# Autodesk Inventor assembly: chassis_2
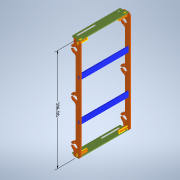
[picture p0: Inventor's stored thumbnail of the model, 180x180]
Saved by Autodesk Inventor 2022 (Build 260153000, 153)
## iProperties
Created: 2023-03-24
Part Number: chassis_2
Document SubType Name: Assembly
Designer: Johnny Jou
Author: Johnny Jou
## Documents named in this file (5)
- C:\Users\Johnny Jou\Documents\GitHub\Areo_Rider_Cabin\car\chassis_2.iam
- C:\Users\Johnny Jou\Documents\GitHub\Areo_Rider_Cabin\car\chassis_1_1.ipt
- C:\Users\Johnny Jou\Documents\GitHub\Areo_Rider_Cabin\car\chassis_1_2.ipt
- C:\Users\Johnny Jou\Documents\GitHub\Areo_Rider_Cabin\car\chassis_1_3.ipt
- C:\Users\Johnny Jou\Documents\GitHub\Areo_Rider_Cabin\car\chassis_1_4.ipt
## Components (10 placed, 4 different names)
1. chassis_1_1:1 — 貼合:1, 齊平:1, 齊平:2, 貼合:3, 貼合:4, 貼合:6, 齊平:5, 貼合:7, 貼合:8, 齊平:6, 貼合:9, 齊平:8, 齊平:12
2. chassis_1_1:2 — 貼合:2, 貼合:5, 齊平:4, 齊平:9, 齊平:15
3. chassis_1_2:1 — 貼合:1, 齊平:2, 齊平:3, 貼合:10, 齊平:7, 齊平:10
4. chassis_1_2:2 — 貼合:2, 齊平:1, 齊平:3, 貼合:3, 貼合:4, 貼合:5, 齊平:4, 貼合:11, 齊平:13, 齊平:16
5. chassis_1_3:1 — 貼合:6, 齊平:5, 貼合:7
6. chassis_1_3:2 — 貼合:8, 齊平:6, 貼合:9
7. chassis_1_4:1 — 貼合:10, 齊平:7, 齊平:8, 齊平:11
8. chassis_1_4:2 — 齊平:9, 齊平:10, 齊平:11
9. chassis_1_4:3 — 貼合:11, 齊平:12, 齊平:13, 齊平:14
10. chassis_1_4:4 — 齊平:14, 齊平:15, 齊平:16
## Relationships (27: Flush 16, Mate 11)
- 貼合:1 [Mate]: chassis_1_1:1 ↔ chassis_1_2:1
- 貼合:2 [Mate]: chassis_1_1:2 ↔ chassis_1_2:2
- 齊平:1 [Flush]: chassis_1_1:1 ↔ chassis_1_2:2
- 齊平:2 [Flush]: chassis_1_1:1 ↔ chassis_1_2:1
- 齊平:3 [Flush]: chassis_1_2:1 ↔ chassis_1_2:2
- 貼合:3 [Mate]: chassis_1_1:1 ↔ chassis_1_2:2
- 貼合:4 [Mate]: chassis_1_1:1 ↔ chassis_1_2:2
- 貼合:5 [Mate]: chassis_1_1:2 ↔ chassis_1_2:2
- 齊平:4 [Flush]: chassis_1_1:2 ↔ chassis_1_2:2
- 貼合:6 [Mate]: chassis_1_1:1 ↔ chassis_1_3:1
- 齊平:5 [Flush]: chassis_1_1:1 ↔ chassis_1_3:1
- 貼合:7 [Mate]: chassis_1_1:1 ↔ chassis_1_3:1
- 貼合:8 [Mate]: chassis_1_1:1 ↔ chassis_1_3:2
- 齊平:6 [Flush]: chassis_1_1:1 ↔ chassis_1_3:2
- 貼合:9 [Mate]: chassis_1_1:1 ↔ chassis_1_3:2
- 貼合:10 [Mate]: chassis_1_2:1 ↔ chassis_1_4:1
- 齊平:7 [Flush]: chassis_1_2:1 ↔ chassis_1_4:1
- 齊平:8 [Flush]: chassis_1_1:1 ↔ chassis_1_4:1
- 齊平:9 [Flush]: chassis_1_1:2 ↔ chassis_1_4:2
- 齊平:10 [Flush]: chassis_1_2:1 ↔ chassis_1_4:2
- 齊平:11 [Flush]: chassis_1_4:1 ↔ chassis_1_4:2
- 貼合:11 [Mate]: chassis_1_2:2 ↔ chassis_1_4:3
- 齊平:12 [Flush]: chassis_1_1:1 ↔ chassis_1_4:3
- 齊平:13 [Flush]: chassis_1_2:2 ↔ chassis_1_4:3
- 齊平:14 [Flush]: chassis_1_4:3 ↔ chassis_1_4:4
- 齊平:15 [Flush]: chassis_1_1:2 ↔ chassis_1_4:4
- 齊平:16 [Flush]: chassis_1_2:2 ↔ chassis_1_4:4
